# Autodesk Inventor assembly: LedRow
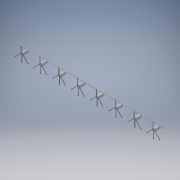
[picture p0: Inventor's stored thumbnail of the model, 180x180]
Saved by Autodesk Inventor 2019.3 (Build 233278000, 278)
## iProperties
Created: 2019-01-08
Part Number: LedRow
Material: Generisch
Document SubType Name: Assembly
Designer: Jonas
Author: Jonas
## Documents named in this file (3)
- C:\Users\Jonas\Desktop\RGBCube\RGBCubev2\CAD\Led\LedRow.iam
- C:\Users\Jonas\Desktop\RGBCube\RGBCubev2\CAD\Led\RGBLed bent.iam
- C:\Users\Jonas\Desktop\RGBCube\RGBCubev2\CAD\Led\WireCathode.ipt
## Components (9 placed, 2 different names)
1. RGBLed bent:5 [sub-assembly] — Einfügen:6, Passend:1
2. RGBLed bent:6 [sub-assembly] — Einfügen:5, Passend:3
3. RGBLed bent:7 [sub-assembly] — Einfügen:4, Passend:2
4. RGBLed bent:8 [sub-assembly] — Einfügen:7, Passend:4
5. WireCathode:1 — Einfügen:4, Einfügen:5, Einfügen:6, Einfügen:7, Einfügen:8, Einfügen:9, Einfügen:10, Einfügen:11
6. RGBLed bent:9 [sub-assembly] — Einfügen:8, Passend:5
7. RGBLed bent:10 [sub-assembly] — Einfügen:9, Passend:6
8. RGBLed bent:11 [sub-assembly] — Einfügen:10, Passend:7
9. RGBLed bent:12 [sub-assembly] — Einfügen:11, Passend:8
## Relationships (16: Insert 8, Mate 8)
- Einfügen:4 [Insert] (50 mm): RGBLed bent:7 ↔ WireCathode:1
- Einfügen:5 [Insert] (80 mm): RGBLed bent:6 ↔ WireCathode:1
- Einfügen:6 [Insert] (20 mm): RGBLed bent:5 ↔ WireCathode:1
- Einfügen:7 [Insert] (110 mm): RGBLed bent:8 ↔ WireCathode:1
- Einfügen:8 [Insert] (140 mm): WireCathode:1 ↔ RGBLed bent:9
- Einfügen:9 [Insert] (170 mm): WireCathode:1 ↔ RGBLed bent:10
- Einfügen:10 [Insert] (200 mm): WireCathode:1 ↔ RGBLed bent:11
- Einfügen:11 [Insert] (230 mm): WireCathode:1 ↔ RGBLed bent:12
- Passend:1 [Mate]: RGBLed bent:5
- Passend:2 [Mate]: RGBLed bent:7
- Passend:3 [Mate]: RGBLed bent:6
- Passend:4 [Mate]: RGBLed bent:8
- Passend:5 [Mate]: RGBLed bent:9
- Passend:6 [Mate]: RGBLed bent:10
- Passend:7 [Mate]: RGBLed bent:11
- Passend:8 [Mate]: RGBLed bent:12
